# Autodesk Inventor assembly: DriveChain2
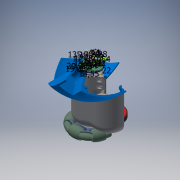
[picture p0: Inventor's stored thumbnail of the model, 180x180]
Saved by Autodesk Inventor 2019.1 (Build 231200000, 200)
## iProperties
Created: 2018-07-27
Part Number: DriveChain2
Material: Generisch
Document SubType Name: Assembly
Designer: JochenAlt
Author: JochenAlt
## Documents named in this file (11)
- D:\Projects\Ondine\CAD\DriveChain.iam
- D:\Projects\Ondine\CAD\BushOmniWheel.ipt
- D:\Projects\Ondine\CAD\DriveChainEnclosure.ipt
- D:\Projects\Ondine\CAD\BeltDriveAxis.ipt
- D:\Projects\Ondine\CAD\BushBeltDriveTL.ipt
- D:\Projects\Ondine\CAD\Bearings\W 637_4 X-2Z.iam
- D:\Projects\Ondine\CAD\OmniWheel.iam
- D:\Projects\Ondine\CAD\Beltdrive\BeltGear.iam
- D:\Projects\Ondine\CAD\BeltDriveAxisSleeve.ipt
- C:\Users\JochenAlt\Documents\Inventor\Content Center Files\R2019\de-DE\DIN 912\DIN 912 - M2 x 0,4 x 16 x 15.ipt
- C:\Users\JochenAlt\Documents\Inventor\Content Center Files\R2019\de-DE\DIN 934\DIN 934 - M2 x 0,4.ipt
## Components (17 placed, 9 different names)
1. DriveChainEnclosure:1 — Passend:105, Passend:106, Passend:130, Passend:131, Passend:133, Passend:134, Passend:135, Passend:136, Passend:150, Passend:151, Passend:152, Passend:153, Passend:154, Passend:155, Passend:157, Passend:159, Passend:161
2. W 637_4 X-2Z:3 [sub-assembly] — Passend:130, Passend:131
3. W 637_4 X-2Z:1 [sub-assembly] — Passend:105, Passend:106, Passend:119, Passend:140, Passend:149
4. BushOmniWheel:4 — Passend:119, Passend:128, Passend:140
5. BushOmniWheel:3 — Passend:80
6. BeltdriveAxis — Passend:80, Passend:132, Passend:133, Passend:136, Passend:137, Passend:138
7. BushOmniWheel:1 — Passend:147, Passend:148, Passend:149
8. OmniWheel:1 [sub-assembly] — Passend:141, Passend:146, Passend:148
9. W 637_4 X-2Z:4 [sub-assembly] — Passend:132, Passend:134, Passend:135
10. NewBeltGear:1 [sub-assembly] — Passend:128, Passend:137, Passend:139, Passend:141, Passend:146, Passend:147
11. BeltDriveAxisSleeve:1 — Passend:138, Passend:139
12. DIN 912 - ersetzt durch DIN EN ISO 4762 M2 x 16:1 — Passend:150, Passend:151, Passend:158
13. DIN 912 - ersetzt durch DIN EN ISO 4762 M2 x 16:2 — Passend:152, Passend:153, Passend:156
14. DIN 912 - ersetzt durch DIN EN ISO 4762 M2 x 16:3 — Passend:154, Passend:155, Passend:160
15. DIN 934 - ersetzt durch DIN EN 24032/28673/28674 M2:1 — Passend:156, Passend:157
16. DIN 934 - ersetzt durch DIN EN 24032/28673/28674 M2:2 — Passend:158, Passend:159
17. DIN 934 - ersetzt durch DIN EN 24032/28673/28674 M2:3 — Passend:160, Passend:161
## Relationships (33: Mate 33)
- Passend:80 [Mate]: BushOmniWheel:3 ↔ BeltdriveAxis
- Passend:105 [Mate]: DriveChainEnclosure:1 ↔ W 637_4 X-2Z:1
- Passend:106 [Mate]: DriveChainEnclosure:1 ↔ W 637_4 X-2Z:1
- Passend:119 [Mate]: W 637_4 X-2Z:1 ↔ BushOmniWheel:4
- Passend:128 [Mate]: BushOmniWheel:4 ↔ NewBeltGear:1
- Passend:130 [Mate]: DriveChainEnclosure:1 ↔ W 637_4 X-2Z:3
- Passend:131 [Mate]: DriveChainEnclosure:1 ↔ W 637_4 X-2Z:3
- Passend:132 [Mate]: BeltdriveAxis ↔ W 637_4 X-2Z:4
- Passend:133 [Mate]: DriveChainEnclosure:1 ↔ BeltdriveAxis
- Passend:134 [Mate]: DriveChainEnclosure:1 ↔ W 637_4 X-2Z:4
- Passend:135 [Mate]: DriveChainEnclosure:1 ↔ W 637_4 X-2Z:4
- Passend:136 [Mate]: DriveChainEnclosure:1 ↔ BeltdriveAxis
- Passend:137 [Mate]: BeltdriveAxis ↔ NewBeltGear:1
- Passend:138 [Mate]: BeltdriveAxis ↔ BeltDriveAxisSleeve:1
- Passend:139 [Mate]: NewBeltGear:1 ↔ BeltDriveAxisSleeve:1
- Passend:140 [Mate]: W 637_4 X-2Z:1 ↔ BushOmniWheel:4
- Passend:141 [Mate]: OmniWheel:1 ↔ NewBeltGear:1
- Passend:146 [Mate]: OmniWheel:1 ↔ NewBeltGear:1
- Passend:147 [Mate]: BushOmniWheel:1 ↔ NewBeltGear:1
- Passend:148 [Mate]: BushOmniWheel:1 ↔ OmniWheel:1
- Passend:149 [Mate]: W 637_4 X-2Z:1 ↔ BushOmniWheel:1
- Passend:150 [Mate]: DriveChainEnclosure:1 ↔ DIN 912 - ersetzt durch DIN EN ISO 4762 M2 x 16:1
- Passend:151 [Mate]: DriveChainEnclosure:1 ↔ DIN 912 - ersetzt durch DIN EN ISO 4762 M2 x 16:1
- Passend:152 [Mate]: DriveChainEnclosure:1 ↔ DIN 912 - ersetzt durch DIN EN ISO 4762 M2 x 16:2
- Passend:153 [Mate]: DriveChainEnclosure:1 ↔ DIN 912 - ersetzt durch DIN EN ISO 4762 M2 x 16:2
- Passend:154 [Mate]: DriveChainEnclosure:1 ↔ DIN 912 - ersetzt durch DIN EN ISO 4762 M2 x 16:3
- Passend:155 [Mate]: DriveChainEnclosure:1 ↔ DIN 912 - ersetzt durch DIN EN ISO 4762 M2 x 16:3
- Passend:156 [Mate]: DIN 912 - ersetzt durch DIN EN ISO 4762 M2 x 16:2 ↔ DIN 934 - ersetzt durch DIN EN 24032/28673/28674 M2:1
- Passend:157 [Mate]: DriveChainEnclosure:1 ↔ DIN 934 - ersetzt durch DIN EN 24032/28673/28674 M2:1
- Passend:158 [Mate]: DIN 912 - ersetzt durch DIN EN ISO 4762 M2 x 16:1 ↔ DIN 934 - ersetzt durch DIN EN 24032/28673/28674 M2:2
- Passend:159 [Mate]: DriveChainEnclosure:1 ↔ DIN 934 - ersetzt durch DIN EN 24032/28673/28674 M2:2
- Passend:160 [Mate]: DIN 912 - ersetzt durch DIN EN ISO 4762 M2 x 16:3 ↔ DIN 934 - ersetzt durch DIN EN 24032/28673/28674 M2:3
- Passend:161 [Mate]: DriveChainEnclosure:1 ↔ DIN 934 - ersetzt durch DIN EN 24032/28673/28674 M2:3
